# Autodesk Inventor assembly: XT60 Connectors
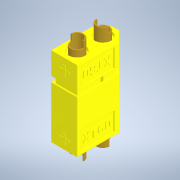
[picture p0: Inventor's stored thumbnail of the model, 180x180]
Saved by Autodesk Inventor 2020.1 (Build 241239000, 239)
## iProperties
Created: 2014-04-12
Part Number: XT60 Connectors
Document SubType Name: Assembly
Designer: Petar
Sending System: Autodesk Inventor 2011
Preprocessor: Autodesk Inventor 2011
Title: C:\Users\Malcolm\Documents\Inventor\RC\XT60 Connectors.stp
Author: Malcolm
## Documents named in this file (3)
- D:\OMG\E-Board\CAD\Inventor\Electrical Components\XT60\XT60 Connectors.iam
- D:\OMG\E-Board\CAD\Inventor\Electrical Components\XT60\XT60 Connector Male Connector.iam
- D:\OMG\E-Board\CAD\Inventor\Electrical Components\XT60\XT60 Connector Female Connector.iam
## Components (2 placed, 2 different names)
1. XT60 Connector Male Connector_1 [sub-assembly] — Rigid:1
2. XT60 Connector Female Connector_1 [sub-assembly] — Rigid:1
## Relationships (1: WeldJoint 1)
- Rigid:1 [WeldJoint]: XT60 Connector Male Connector_1 ↔ XT60 Connector Female Connector_1
